# Autodesk Inventor assembly: CL4-300
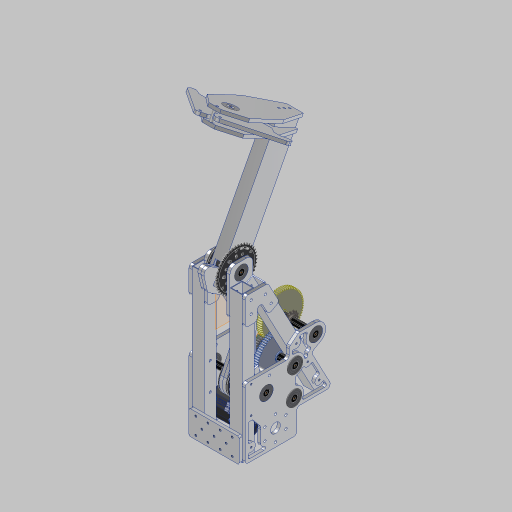
[picture p0: Inventor's stored thumbnail of the model, 512x512]
Saved by Autodesk Inventor 2023.5 (Build 275446000, 446)
## iProperties
Created: 2025-02-04
Part Number: CL4-300
Document SubType Name: Assembly
Designer: brand
Mass: 3247.43 g
Surface Area: 7567.76 cm^2
Volume: 1278.12 cm^3
Density: 2.54079 g/cm^3
Author: brand
## Documents named in this file (8)
- C:\Users\slick\OneDrive\Desktop\2025-ReefScape---CAD\Climber\CL4\CL4-300.iam
- C:\Users\slick\OneDrive\Desktop\2025-ReefScape---CAD\Climber\CL4\CL4-200.iam
- C:\Users\slick\OneDrive\Desktop\2025-ReefScape---CAD\Climber\CL4\CL4-100.iam
- C:\Users\slick\OneDrive\Desktop\2025-ReefScape---CAD\Climber\CL4\CL4-011.ipt
- C:\Users\slick\OneDrive\Desktop\2025-ReefScape---CAD\COMMON PARTS\SPROCKETS\25\WCP-0967 42t 25_chain.ipt
- C:\Users\slick\OneDrive\Desktop\2025-ReefScape---CAD\Climber\CL4\CL4-400-GB.iam
- C:\Users\slick\OneDrive\Desktop\2025-ReefScape---CAD\COMMON PARTS\BEARINGS\0_500_ID_x_1_125_OD_x_0_313_WD_Flanged_Bearing_217-2731.ipt
- C:\Users\slick\OneDrive\Desktop\2025-ReefScape---CAD\Climber\CL4\CL4-021.ipt
## Components (8 placed, 7 different names)
1. CL4-200:1 [sub-assembly] — Angle:1, Insert:6, Insert:7, Insert:8, Insert:9, Insert:10, Insert:11
2. CL4-100:1 [sub-assembly] — Mate:2, Angle:1, Mate:13, Mate:14, Mate:15
3. CL4-011:1 — Mate:2, Mate:19, Flush:2
4. WCP-0967 42t 25_chain:1 — Mate:13, Mate:14, Mate:15, Mate:20
5. CL4-400-GB:1 [sub-assembly] — Insert:8, Insert:9
6. 0_500_ID_x_1_125_OD_x_0_313_WD_Flanged_Bearing_217-2731:1 — Insert:7
7. 0_500_ID_x_1_125_OD_x_0_313_WD_Flanged_Bearing_217-2731:2 — Insert:6, Mate:19, Flush:2, Mate:20
8. CL4-021:1 — Insert:10, Insert:11
## Relationships (14: Mate 6, Insert 6, Angle 1, Flush 1)
- Mate:2: CL4-100:1 ↔ CL4-011:1
- Angle:1 (0 deg): CL4-200:1 ↔ CL4-100:1
- Mate:13: CL4-100:1 ↔ WCP-0967 42t 25_chain:1
- Mate:14: CL4-100:1 ↔ WCP-0967 42t 25_chain:1
- Mate:15: CL4-100:1 ↔ WCP-0967 42t 25_chain:1
- Insert:6: CL4-200:1 ↔ 0_500_ID_x_1_125_OD_x_0_313_WD_Flanged_Bearing_217-2731:2
- Insert:7: CL4-200:1 ↔ 0_500_ID_x_1_125_OD_x_0_313_WD_Flanged_Bearing_217-2731:1
- Mate:19: CL4-011:1 ↔ 0_500_ID_x_1_125_OD_x_0_313_WD_Flanged_Bearing_217-2731:2
- Flush:2: CL4-011:1 ↔ 0_500_ID_x_1_125_OD_x_0_313_WD_Flanged_Bearing_217-2731:2
- Mate:20 (1.5875 mm): WCP-0967 42t 25_chain:1 ↔ 0_500_ID_x_1_125_OD_x_0_313_WD_Flanged_Bearing_217-2731:2
- Insert:8: CL4-200:1 ↔ CL4-400-GB:1
- Insert:9: CL4-200:1 ↔ CL4-400-GB:1
- Insert:10: CL4-200:1 ↔ CL4-021:1
- Insert:11: CL4-200:1 ↔ CL4-021:1
